# Autodesk Inventor assembly: sumec_smd
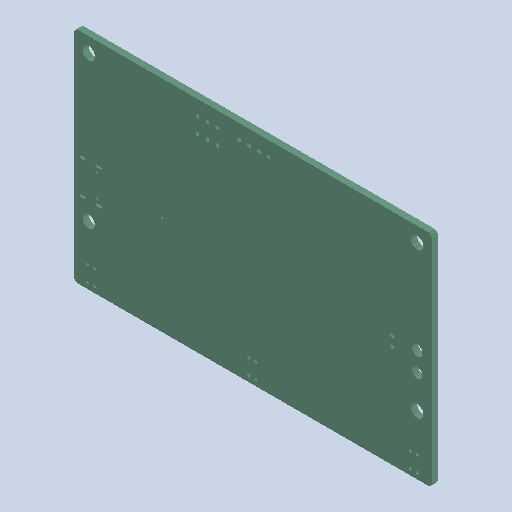
[picture p0: Inventor's stored thumbnail of the model, 512x512]
Saved by Autodesk Inventor 2024 (Build 280153000, 153)
## iProperties
Company: Kicad
Created: 2023-10-31
Part Number: sumec_smd
Description: KiCad electronic assembly
Document SubType Name: Assembly
Designer: Simak
Authority: Unknown
Sending System: KiCad to STEP converter
Preprocessor: Open CASCADE STEP processor 7.6
Title: sumec.step
Author: Pcbnew
## Documents named in this file (16)
- C:\Users\Simak\OneDrive\Dokumenty\GitHub\RoboCop\- 3D -\el._parts\sumec_smd.iam
- C:\Users\Simak\OneDrive\Dokumenty\GitHub\RoboCop\- 3D -\el._parts\sumec\LED_1206_3216Metric.iam
- C:\Users\Simak\OneDrive\Dokumenty\GitHub\RoboCop\- 3D -\el._parts\sumec\R_1206_3216Metric.iam
- C:\Users\Simak\OneDrive\Dokumenty\GitHub\RoboCop\- 3D -\el._parts\sumec\SSOP-24_5.3x8.2mm_P0.65mm.iam
- C:\Users\Simak\OneDrive\Dokumenty\GitHub\RoboCop\- 3D -\el._parts\sumec\SW_SPST_B3U-1000P.iam
- C:\Users\Simak\OneDrive\Dokumenty\GitHub\RoboCop\- 3D -\el._parts\sumec\jst - 1 mm 6 pin female (Å¡patnÃ½).iam
- C:\Users\Simak\OneDrive\Dokumenty\GitHub\RoboCop\- 3D -\el._parts\sumec\TO-252-3_TabPin2.iam
- C:\Users\Simak\OneDrive\Dokumenty\GitHub\RoboCop\- 3D -\el._parts\sumec\H254_90deg_4pin.iam
- C:\Users\Simak\OneDrive\Dokumenty\GitHub\RoboCop\- 3D -\el._parts\sumec\C_1206_3216Metric.iam
- C:\Users\Simak\OneDrive\Dokumenty\GitHub\RoboCop\- 3D -\el._parts\sumec\PinSocket_1x03_P2.54mm_Vertical.iam
- C:\Users\Simak\OneDrive\Dokumenty\GitHub\RoboCop\- 3D -\el._parts\sumec\PinHeader_1x02_P2.54mm_Vertical.iam
- C:\Users\Simak\OneDrive\Dokumenty\GitHub\RoboCop\- 3D -\el._parts\sumec\D_1206_3216Metric.iam
- C:\Users\Simak\OneDrive\Dokumenty\GitHub\RoboCop\- 3D -\el._parts\sumec\TSOT-23-6.iam
- C:\Users\Simak\OneDrive\Dokumenty\GitHub\RoboCop\- 3D -\el._parts\sumec\TYPE-C-31-M-12.iam
- C:\Users\Simak\OneDrive\Dokumenty\GitHub\RoboCop\- 3D -\el._parts\sumec\QRE1113.iam
- C:\Users\Simak\OneDrive\Dokumenty\GitHub\RoboCop\- 3D -\el._parts\sumec_pcb\PCB.ipt
## Components (51 placed, 51 different names)
1. 2 [sub-assembly]
2. 4 [sub-assembly]
3. 5 [sub-assembly]
4. 6 [sub-assembly]
5. 8 [sub-assembly]
6. 10 [sub-assembly]
7. 11 [sub-assembly]
8. 13 [sub-assembly]
9. 17 [sub-assembly]
10. 19 [sub-assembly] — Proti sobě:1, Stejný směr:1, Proti sobě:2
11. 20 [sub-assembly]
12. 21 [sub-assembly]
13. 22 [sub-assembly]
14. 23 [sub-assembly]
15. 25 [sub-assembly]
16. 27 [sub-assembly]
17. 29 [sub-assembly]
18. 31 [sub-assembly]
19. 32 [sub-assembly]
20. 34 [sub-assembly]
21. 35 [sub-assembly]
22. 36 [sub-assembly]
23. 37 [sub-assembly]
24. 38 [sub-assembly]
25. 39 [sub-assembly]
26. 40 [sub-assembly]
27. 41 [sub-assembly]
28. 42 [sub-assembly]
29. 43 [sub-assembly]
30. 44 [sub-assembly]
31. 45 [sub-assembly]
32. 46 [sub-assembly]
33. 48 [sub-assembly]
34. 49 [sub-assembly]
35. 50 [sub-assembly]
36. 51 [sub-assembly]
37. 52 [sub-assembly]
38. 54 [sub-assembly]
39. 55 [sub-assembly]
40. 56 [sub-assembly]
41. 57 [sub-assembly]
42. 58 [sub-assembly]
43. 59 [sub-assembly]
44. 60 [sub-assembly]
45. 61 [sub-assembly]
46. 62 [sub-assembly]
47. 63 [sub-assembly]
48. 64 [sub-assembly]
49. 65 [sub-assembly]
50. 66 [sub-assembly]
51. 67 — Proti sobě:1, Stejný směr:1, Proti sobě:2
## Relationships (3: Mate 2, Flush 1)
- Proti sobě:1 [Mate]: 19 ↔ 67
- Stejný směr:1 [Flush]: 19 ↔ 67
- Proti sobě:2 [Mate]: 19 ↔ 67
